# Autodesk Inventor assembly: washing_assembly
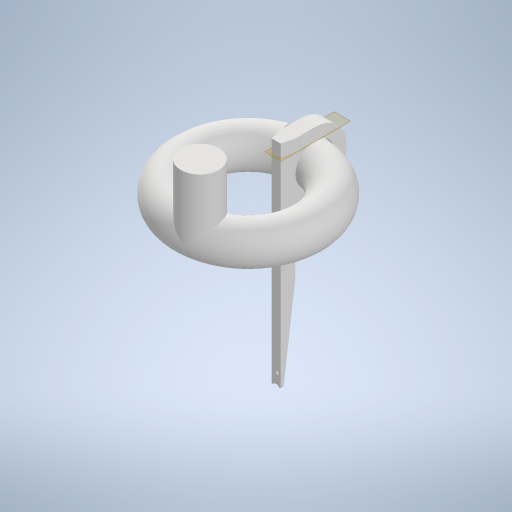
[picture p0: Inventor's stored thumbnail of the model, 512x512]
Saved by Autodesk Inventor 2023.3 (Build 273359000, 359)
## iProperties
Created: 2023-11-29
Part Number: washing_assembly
Document SubType Name: Assembly
Designer: mmelin
Author: mmelin
## Documents named in this file (3)
- X:\chronic_holder\NP2\washing\washing_assembly.iam
- X:\chronic_holder\NP2\washing\np2_washing_arm.ipt
- X:\chronic_holder\NP2\washing\wash_ring.ipt
## Components (2 placed, 2 different names)
1. np2_washing_arm:1 — Angle:1, Tangent:1
2. wash_ring:1 — Flush:1
## Relationships (3: Angle 1, Tangent 1, Flush 1)
- Angle:1 (0 deg): np2_washing_arm:1
- Tangent:1: np2_washing_arm:1
- Flush:1: wash_ring:1
